# Autodesk Inventor assembly: body_assembly
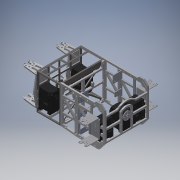
[picture p0: Inventor's stored thumbnail of the model, 180x180]
Saved by Autodesk Inventor 2018 (Build 220112000, 112)
## iProperties
Created: 2018-11-26
Part Number: body_assembly
Document SubType Name: Assembly
Designer: bitbots
Mass: 613.238 g
Surface Area: 2643.37 cm^2
Volume: 613.238 cm^3
Density: 1 g/cm^3
Author: bitbots
## Documents named in this file (4)
- C:\Users\jaspe\bitbots_hardware\wolfgang\assembly\body\body_assembly.iam
- C:\Users\jaspe\bitbots_hardware\wolfgang\assembly\body\hip_connector.ipt
- C:\Users\jaspe\bitbots_hardware\wolfgang\assembly\body\shoulder_connector.ipt
- C:\Users\jaspe\bitbots_hardware\wolfgang\assembly\body\torso_link.iam
## Components (5 placed, 3 different names)
1. hip_connector:1 — Mate:10, Mate:11, Mate:12
2. hip_connector:2 — Mate:7, Mate:8, Mate:9
3. shoulder_connector:1 — Mate:4, Mate:5, Mate:6
4. shoulder_connector:2 — Mate:1, Mate:2, Mate:3
5. torso_link:1 [sub-assembly] — Mate:1, Mate:2, Mate:3, Mate:4, Mate:5, Mate:6, Mate:7, Mate:8, Mate:9, Mate:10, Mate:11, Mate:12
## Relationships (12: Mate 12)
- Mate:1: shoulder_connector:2 ↔ torso_link:1
- Mate:2: shoulder_connector:2 ↔ torso_link:1
- Mate:3: shoulder_connector:2 ↔ torso_link:1
- Mate:4: shoulder_connector:1 ↔ torso_link:1
- Mate:5: shoulder_connector:1 ↔ torso_link:1
- Mate:6: shoulder_connector:1 ↔ torso_link:1
- Mate:7: hip_connector:2 ↔ torso_link:1
- Mate:8: hip_connector:2 ↔ torso_link:1
- Mate:9: hip_connector:2 ↔ torso_link:1
- Mate:10: hip_connector:1 ↔ torso_link:1
- Mate:11: hip_connector:1 ↔ torso_link:1
- Mate:12: hip_connector:1 ↔ torso_link:1
